# Autodesk Inventor assembly: Assembly1
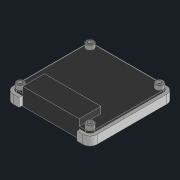
[picture p0: Inventor's stored thumbnail of the model, 180x180]
Saved by Autodesk Inventor 2022 (Build 260153000, 153)
## iProperties
Created: 2021-09-16
Part Number: Assembly1
Document SubType Name: Assembly
Designer: Yuta Kage
Author: Yuta Kage
## Documents named in this file (5)
- C:\Users\yuta0\Documents\GitHub\catchrobo_hardware\assy-robot\Assembly1.iam
- C:\Users\yuta0\Documents\GitHub\catchrobo_hardware\assy-robot\base47.ipt
- C:\Users\yuta0\Documents\GitHub\zebra_hardware\hardware\zebra_cad_v1.0\driver_ver1.0.ipt
- C:\Users\yuta0\Documents\GitHub\catchrobo_hardware\assy-robot\LBNR3.ipt
- C:\Users\yuta0\Documents\GitHub\catchrobo_hardware\assy-robot\CB3-6.ipt
## Components (10 placed, 4 different names)
1. base47:1 — メイト:4, 角度:1, メイト:5, メイト:6, メイト:7, メイト:8
2. driver_ver1.0:1 — メイト:6, メイト:7, メイト:8, メイト:9, メイト:10
3. CB3-6:1 — メイト:9, メイト:10
4. LBNR3:1 — メイト:4, 角度:1, メイト:5
5. CB3-6:2
6. LBNR3:2
7. CB3-6:3
8. LBNR3:3
9. CB3-6:4
10. LBNR3:4
## Component patterns: (4 elements, first: CB3-6:1 + LBNR3:1)
## Relationships (8: Mate 7, Angle 1)
- メイト:4 [Mate]: base47:1 ↔ LBNR3:1
- 角度:1 [Angle] (0 deg): base47:1 ↔ LBNR3:1
- メイト:5 [Mate]: base47:1 ↔ LBNR3:1
- メイト:6 [Mate]: base47:1 ↔ driver_ver1.0:1
- メイト:7 [Mate]: base47:1 ↔ driver_ver1.0:1
- メイト:8 [Mate]: base47:1 ↔ driver_ver1.0:1
- メイト:9 [Mate]: driver_ver1.0:1 ↔ CB3-6:1
- メイト:10 [Mate]: driver_ver1.0:1 ↔ CB3-6:1
